# Autodesk Inventor assembly: Zespół
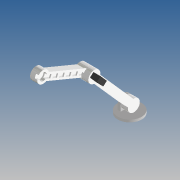
[picture p0: Inventor's stored thumbnail of the model, 180x180]
Saved by Autodesk Inventor 2022.3 (Build 263350000, 350)
## iProperties
Created: 2023-06-25
Part Number: Zespół
Document SubType Name: Assembly
Designer: Chyba Ja
Author: Chyba Ja
## Documents named in this file (5)
- C:\Users\Chyba Ja\Documents\Inventor\WALL-E\Zespół.iam
- C:\Users\Chyba Ja\Documents\Inventor\WALL-E\1stopien.ipt
- C:\Users\Chyba Ja\Documents\Inventor\WALL-E\2stopien.ipt
- C:\Users\Chyba Ja\Documents\Inventor\WALL-E\podstawa.ipt
- C:\Users\Chyba Ja\Documents\Inventor\WALL-E\serwo.ipt
## Components (4 placed, 4 different names)
1. 1stopien:1 — Zestawiające:1, Zestawiające:2, Zestawiające:5, Zestawiające:6, Zestawiające:7, Zestawiające:9
2. 2stopien:1 — Zestawiające:7, Zestawiające:8
3. podstawa:1 — Zestawiające:1, Zestawiające:2
4. serwo:1 — Zestawiające:5, Zestawiające:6, Zestawiające:8, Zestawiające:9
## Relationships (7: Mate 7)
- Zestawiające:1 [Mate]: 1stopien:1 ↔ podstawa:1
- Zestawiające:2 [Mate]: 1stopien:1 ↔ podstawa:1
- Zestawiające:5 [Mate]: 1stopien:1 ↔ serwo:1
- Zestawiające:6 [Mate]: 1stopien:1 ↔ serwo:1
- Zestawiające:7 [Mate]: 1stopien:1 ↔ 2stopien:1
- Zestawiające:8 [Mate]: 2stopien:1 ↔ serwo:1
- Zestawiające:9 [Mate]: 1stopien:1 ↔ serwo:1
